# Autodesk Inventor assembly: CardPower
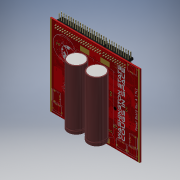
[picture p0: Inventor's stored thumbnail of the model, 180x180]
Saved by Autodesk Inventor 2017 (Build 210142000, 142)
## iProperties
Created: 2017-10-19
Part Number: CardPower
Document SubType Name: Assembly
Designer: Bradley
Author: Bradley
## Documents named in this file (4)
- C:\Users\Bradley\Desktop\CougSat\CubeSatCardGuides\CardPower\CardPower.iam
- C:\Users\Bradley\Desktop\CougSat\CubeSatCardGuides\Components\CougSatBus_Male.iam
- C:\Users\Bradley\Desktop\CougSat\CubeSatCardGuides\CardPower\CardPower_PCB.ipt
- C:\Users\Bradley\Desktop\CougSat\CubeSatCardGuides\Components\Battery_18650.ipt
## Components (4 placed, 3 different names)
1. CardPower_PCB:1 — Mate:1, Mate:2, Mate:3, Mate:4, Mate:5, Mate:6
2. CougSatBus_Male:1 [sub-assembly] — Mate:1, Mate:2, Mate:3, Mate:4
3. Battery_18650:1 — Mate:5, Flush:1, Mate:7
4. Battery_18650:2 — Mate:6, Flush:2, Mate:8
## Relationships (10: Mate 8, Flush 2)
- Mate:1: CardPower_PCB:1 ↔ CougSatBus_Male:1
- Mate:2 (-0.3111 mm): CardPower_PCB:1 ↔ CougSatBus_Male:1
- Mate:3 (-0.3111 mm): CardPower_PCB:1 ↔ CougSatBus_Male:1
- Mate:4 (-0.3111 mm): CardPower_PCB:1 ↔ CougSatBus_Male:1
- Mate:5 (9 mm): CardPower_PCB:1 ↔ Battery_18650:1
- Mate:6 (9 mm): CardPower_PCB:1 ↔ Battery_18650:2
- Flush:1 (11 mm): Battery_18650:1
- Flush:2 (-11 mm): Battery_18650:2
- Mate:7 (-42 mm): Battery_18650:1
- Mate:8 (-42 mm): Battery_18650:2
